# Autodesk Inventor assembly: Tweepr
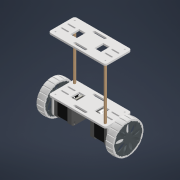
[picture p0: Inventor's stored thumbnail of the model, 180x180]
Saved by Autodesk Inventor 2022.1 (Build 261234000, 234)
## iProperties
Created: 2021-10-11
Part Number: Tweepr
Document SubType Name: Assembly
Designer: Santiago Martínez
Mass: 278.235 g
Surface Area: 1464.6 cm^2
Volume: 254.498 cm^3
Density: 1.09327 g/cm^3
Author: Santiago Martínez
## Documents named in this file (7)
- D:\Santiago\Documents\My Works\Universidad de Los Andes\Proyecto de Grado IELE\Tweepr\3- CAD\Tweepr.iam
- D:\Santiago\Documents\My Works\Universidad de Los Andes\Proyecto de Grado IELE\Tweepr\3- CAD\Base.ipt
- D:\Santiago\Documents\My Works\Universidad de Los Andes\Proyecto de Grado IELE\Tweepr\3- CAD\Standart Parts\Nema 17 Stepper (17HS4401)17HS4401 Nema 17 Stepper.iam
- D:\Santiago\Documents\My Works\Universidad de Los Andes\Proyecto de Grado IELE\Tweepr\3- CAD\Brass Spacer.ipt
- D:\Santiago\Documents\My Works\Universidad de Los Andes\Proyecto de Grado IELE\Tweepr\3- CAD\Top.ipt
- D:\Santiago\Documents\My Works\Universidad de Los Andes\Proyecto de Grado IELE\Tweepr\3- CAD\Wheel Outer.ipt
- D:\Santiago\Documents\My Works\Universidad de Los Andes\Proyecto de Grado IELE\Tweepr\3- CAD\Wheel Inside.ipt
## Components (12 placed, 6 different names)
1. Base:1 — Mate:1, Mate:2, Mate:3, Mate:4, Mate:5, Mate:6, Mate:7, Mate:8, Mate:9, Mate:11, Mate:15, Mate:16, Angle:2, Angle:3, Angle:5, Angle:6
2. Nema 17 Stepper (17HS4401)17HS4401 Nema 17 Stepper:1 [sub-assembly] — Mate:5, Mate:6, Mate:7, Mate:8, Mate:22, Mate:23
3. Nema 17 Stepper (17HS4401)17HS4401 Nema 17 Stepper:2 [sub-assembly] — Mate:1, Mate:2, Mate:3, Mate:4, Mate:24, Mate:25
4. Brass Spacer:1 — Mate:11, Mate:16, Angle:2, Mate:20, Mate:28, Flush:3, Mate:29
5. Brass Spacer:3 — Mate:9, Mate:15, Angle:3, Mate:17, Mate:30, Flush:4, Mate:31
6. Top:1 — Mate:17, Mate:20, Mate:32
7. Wheel Inside:1 — Mate:22, Mate:23, Angle:6, Mate:26, Flush:1
8. Wheel Inside:2 — Mate:24, Mate:25, Angle:5, Mate:27, Flush:2
9. Wheel Outer:1 — Mate:27, Flush:2
10. Wheel Outer:2 — Mate:26, Flush:1
11. Brass Spacer:4 — Mate:28, Flush:3, Mate:29
12. Brass Spacer:5 — Mate:30, Flush:4, Mate:31, Mate:32
## Relationships (33: Mate 25, Angle 4, Flush 4)
- Mate:1: Base:1 ↔ Nema 17 Stepper (17HS4401)17HS4401 Nema 17 Stepper:2
- Mate:2: Base:1 ↔ Nema 17 Stepper (17HS4401)17HS4401 Nema 17 Stepper:2
- Mate:3: Base:1 ↔ Nema 17 Stepper (17HS4401)17HS4401 Nema 17 Stepper:2
- Mate:4: Base:1 ↔ Nema 17 Stepper (17HS4401)17HS4401 Nema 17 Stepper:2
- Mate:5: Base:1 ↔ Nema 17 Stepper (17HS4401)17HS4401 Nema 17 Stepper:1
- Mate:6: Base:1 ↔ Nema 17 Stepper (17HS4401)17HS4401 Nema 17 Stepper:1
- Mate:7: Base:1 ↔ Nema 17 Stepper (17HS4401)17HS4401 Nema 17 Stepper:1
- Mate:8: Base:1 ↔ Nema 17 Stepper (17HS4401)17HS4401 Nema 17 Stepper:1
- Mate:9: Base:1 ↔ Brass Spacer:3
- Mate:11: Base:1 ↔ Brass Spacer:1
- Mate:15: Base:1 ↔ Brass Spacer:3
- Mate:16: Base:1 ↔ Brass Spacer:1
- Angle:2 (0 deg): Base:1 ↔ Brass Spacer:1
- Angle:3 (0 deg): Base:1 ↔ Brass Spacer:3
- Mate:17: Brass Spacer:3 ↔ Top:1
- Mate:20: Brass Spacer:1 ↔ Top:1
- Mate:22: Nema 17 Stepper (17HS4401)17HS4401 Nema 17 Stepper:1 ↔ Wheel Inside:1
- Mate:23: Nema 17 Stepper (17HS4401)17HS4401 Nema 17 Stepper:1 ↔ Wheel Inside:1
- Mate:24: Nema 17 Stepper (17HS4401)17HS4401 Nema 17 Stepper:2 ↔ Wheel Inside:2
- Mate:25: Nema 17 Stepper (17HS4401)17HS4401 Nema 17 Stepper:2 ↔ Wheel Inside:2
- Angle:5 (0 deg): Base:1 ↔ Wheel Inside:2
- Angle:6 (0 deg): Base:1 ↔ Wheel Inside:1
- Mate:26: Wheel Inside:1 ↔ Wheel Outer:2
- Flush:1: Wheel Inside:1 ↔ Wheel Outer:2
- Mate:27: Wheel Inside:2 ↔ Wheel Outer:1
- Flush:2: Wheel Inside:2 ↔ Wheel Outer:1
- Mate:28: Brass Spacer:1 ↔ Brass Spacer:4
- Flush:3: Brass Spacer:1 ↔ Brass Spacer:4
- Mate:29: Brass Spacer:1 ↔ Brass Spacer:4
- Mate:30: Brass Spacer:3 ↔ Brass Spacer:5
- Flush:4: Brass Spacer:3 ↔ Brass Spacer:5
- Mate:31: Brass Spacer:3 ↔ Brass Spacer:5
- Mate:32: Top:1 ↔ Brass Spacer:5
